# Autodesk Inventor assembly: piston
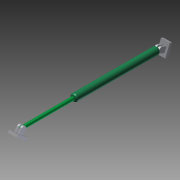
[picture p0: Inventor's stored thumbnail of the model, 180x180]
Saved by Autodesk Inventor 2012 (Build 160160000, 160)
## iProperties
Created: 2011-12-02
Part Number: piston
Document SubType Name: Assembly
Designer: Antonella
Author: Antonella
## Documents named in this file (4)
- C:\Users\Antonella\Documents\GCC Robotics 2012 - Mechanical\Robot 2.0\Weatherproofing Shell\piston.iam
- C:\Users\Antonella\Documents\GCC Robotics 2012 - Mechanical\Robot 2.0\Weatherproofing Shell\piston_outer.ipt
- C:\Users\Antonella\Documents\GCC Robotics 2012 - Mechanical\Robot 2.0\Weatherproofing Shell\piston core.ipt
- C:\Users\Antonella\Documents\GCC Robotics 2012 - Mechanical\Robot 2.0\Weatherproofing Shell\piston mount bracket.ipt
## Components (4 placed, 3 different names)
1. piston_outer:1 — Mate:1, Mate:2, Mate:3, Mate:6
2. piston core:1 — Mate:1, Mate:4, Mate:5, Mate:6
3. piston mount bracket:1 — Mate:2, Mate:3
4. piston mount bracket:2 — Mate:4, Mate:5
## Relationships (6: Mate 6)
- Mate:1: piston_outer:1 ↔ piston core:1
- Mate:2: piston_outer:1 ↔ piston mount bracket:1
- Mate:3: piston_outer:1 ↔ piston mount bracket:1
- Mate:4: piston core:1 ↔ piston mount bracket:2
- Mate:5: piston core:1 ↔ piston mount bracket:2
- Mate:6: piston_outer:1 ↔ piston core:1
